# Autodesk Inventor assembly: TEST-MODULE-CONJUNTO
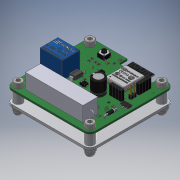
[picture p0: Inventor's stored thumbnail of the model, 180x180]
Saved by Autodesk Inventor 2018.3 (Build 223284000, 284)
## iProperties
Created: 2021-05-04
Part Number: TEST-MODULE-CONJUNTO
Document SubType Name: Assembly
Designer: laguerre
AI: -
B: -
BO: -
BOB: -
BR: -
CCB: -
CCC: -
CO: -
COB: -
COC: -
CR: -
CRB: -
DES: -
GL: -
GLO: -
LA: -
LC: -
LG: -
LGO: -
Linea: -
LT: -
LTC: -
LTO: -
Maquina: -
N: -
NG: -
OBR: -
OBR1: -
OOB: -
OR: -
PC: -
PE: -
PL: -
PO: -
POP: -
QL: -
QLC: -
QLO: -
QR: -
QS: -
QSC: -
QSO: -
RPC: -
RU: -
Sector: -
SG: -
SGO: -
ST: -
STC: -
STO: -
Author: laguerre
## Documents named in this file (8)
- C:\Proyectos\BURN-IN-TEST\TEST-MODULE\3D\TEST-MODULE-ECO.iam
- C:\Proyectos\BURN-IN-TEST\TEST-MODULE\3D\CF-TCA-0001.ipt
- C:\Proyectos\BURN-IN-TEST\TEST-MODULE\3D\PP-LAS-0001.ipt
- C:\Proyectos\BURN-IN-TEST\TEST-MODULE\3D\CF-TCA-0003.ipt
- C:\Proyectos\BURN-IN-TEST\TEST-MODULE\3D\CF-TOR-0002.ipt
- C:\Proyectos\BURN-IN-TEST\TEST-MODULE\3D\CE-IMP-0001.ipt
- C:\Proyectos\BURN-IN-TEST\TEST-MODULE\3D\CF-TOR-0003.ipt
- C:\Proyectos\BURN-IN-TEST\TEST-MODULE\3D\PP-I3D-0002.ipt
## Components (18 placed, 7 different names)
1. PP-LAS-0001:1 — Coincidencia:14, Nivelación:1, Coincidencia:15, Insertar:21, Insertar:22, Insertar:23, Insertar:24, Insertar:33, Insertar:34, Insertar:35, Insertar:36, Nivelación:3
2. DIN 1587 M4:5 — Insertar:22
3. DIN 1587 M4:6 — Insertar:24
4. DIN 1587 M4:7 — Insertar:23
5. DIN 1587 M4:8 — Insertar:21
6. CF-TCA-0001:3 — Insertar:35
7. CF-TCA-0001:4 — Insertar:36
8. ISO 7380-1 M3 x 8:3 — Insertar:34
9. ISO 7380-1 M3 x 8:4 — Insertar:33
10. CE-IMP-0001:1 — Coincidencia:19, Nivelación:2, Nivelación:3, Insertar:37, Insertar:38, Insertar:39, Insertar:40, Insertar:45, Insertar:46, Insertar:47, Insertar:48
11. DIN 912 - reemplazado por DIN EN ISO 4762 M4 x 16:1 — Insertar:37
12. DIN 912 - reemplazado por DIN EN ISO 4762 M4 x 16:2 — Insertar:38
13. DIN 912 - reemplazado por DIN EN ISO 4762 M4 x 16:3 — Insertar:40
14. DIN 912 - reemplazado por DIN EN ISO 4762 M4 x 16:4 — Insertar:39
15. PP-I3D-0002:1 — Insertar:45
16. PP-I3D-0002:2 — Insertar:46
17. PP-I3D-0002:3 — Insertar:48
18. PP-I3D-0002:4 — Insertar:47
## Relationships (22: Insert 16, Mate 3, Flush 3)
- Coincidencia:14 [Mate]: PP-LAS-0001:1
- Nivelación:1 [Flush]: PP-LAS-0001:1
- Coincidencia:15 [Mate]: PP-LAS-0001:1
- Insertar:21: PP-LAS-0001:1 ↔ DIN 1587 M4:8
- Insertar:22: PP-LAS-0001:1 ↔ DIN 1587 M4:5
- Insertar:23: PP-LAS-0001:1 ↔ DIN 1587 M4:7
- Insertar:24: PP-LAS-0001:1 ↔ DIN 1587 M4:6
- Insertar:33: PP-LAS-0001:1 ↔ ISO 7380-1 M3 x 8:4
- Insertar:34: PP-LAS-0001:1 ↔ ISO 7380-1 M3 x 8:3
- Insertar:35: PP-LAS-0001:1 ↔ CF-TCA-0001:3
- Insertar:36: PP-LAS-0001:1 ↔ CF-TCA-0001:4
- Coincidencia:19 [Mate]: CE-IMP-0001:1
- Nivelación:2 [Flush]: CE-IMP-0001:1
- Nivelación:3 [Flush]: PP-LAS-0001:1 ↔ CE-IMP-0001:1
- Insertar:37: CE-IMP-0001:1 ↔ DIN 912 - reemplazado por DIN EN ISO 4762 M4 x 16:1
- Insertar:38: CE-IMP-0001:1 ↔ DIN 912 - reemplazado por DIN EN ISO 4762 M4 x 16:2
- Insertar:39: CE-IMP-0001:1 ↔ DIN 912 - reemplazado por DIN EN ISO 4762 M4 x 16:4
- Insertar:40: CE-IMP-0001:1 ↔ DIN 912 - reemplazado por DIN EN ISO 4762 M4 x 16:3
- Insertar:45: CE-IMP-0001:1 ↔ PP-I3D-0002:1
- Insertar:46: CE-IMP-0001:1 ↔ PP-I3D-0002:2
- Insertar:47: CE-IMP-0001:1 ↔ PP-I3D-0002:4
- Insertar:48: CE-IMP-0001:1 ↔ PP-I3D-0002:3
